# Autodesk Inventor assembly: GabelTop_Link_COG
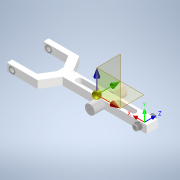
[picture p0: Inventor's stored thumbnail of the model, 180x180]
Saved by Autodesk Inventor 2022 (Build 260153000, 153)
## iProperties
Created: 2022-10-18
Part Number: GabelTop_Link_COG
Document SubType Name: Assembly
Designer: alexw
Mass: 378.635 g
Surface Area: 728.449 cm^2
Volume: 214.913 cm^3
Density: 1.7618 g/cm^3
Author: alexw
## Documents named in this file (5)
- C:\Users\alexw\Documents\Inventor\Projects\03_CurrentProjects\MasterThesis\PSM_V1_Rillenkugellager\COG\GabelTop_Link_COG.iam
- C:\Users\alexw\Documents\Inventor\Projects\03_CurrentProjects\MasterThesis\PSM_V1_Rillenkugellager\Adaptationhorizontalachse_Assembly_Rillenkugellager.iam
- C:\Users\alexw\Documents\Inventor\Projects\03_CurrentProjects\MasterThesis\PSM_V1_Rillenkugellager\SpringCompensation_Outside_SupportPart.ipt
- C:\Users\alexw\Documents\Inventor\Projects\03_CurrentProjects\MasterThesis\PSM_V1_Rillenkugellager\SpringCompensation_Outside_SupportPart_Zwischenstueck.ipt
- C:\Users\alexw\Documents\Inventor\Projects\03_CurrentProjects\MasterThesis\PSM_V1_Rillenkugellager\ContentCenter\de-DE\ISO 4762(2)\ISO 4762 - M10 x 20ISO.ipt
## Components (7 placed, 4 different names)
1. Adaptationhorizontalachse_Assembly_Rillenkugellager:1 [sub-assembly] — Passend:9, Passend:10, Winkel:1, Passend:11, Passend:12, Passend:13, Passend:14, Passend:15, Passend:16, Passend:18
2. SpringCompensation_Outside_SupportPart:1 — Passend:20, Passend:21
3. SpringCompensation_Outside_SupportPart_Zwischenstueck:1 — Passend:12, Passend:13, Passend:17, Passend:20, Passend:21
4. SpringCompensation_Outside_SupportPart_Zwischenstueck:2 — Passend:14, Passend:15, Passend:19, Passend:22, Passend:23
5. ISO 4762 M10 x 20:1 — Passend:16, Passend:17
6. ISO 4762 M10 x 20:2 — Passend:18, Passend:19
7. SpringCompensation_Outside_SupportPart:2 — Passend:22, Passend:23
## Relationships (16: Mate 15, Angle 1)
- Passend:9 [Mate]: Adaptationhorizontalachse_Assembly_Rillenkugellager:1
- Passend:10 [Mate]: Adaptationhorizontalachse_Assembly_Rillenkugellager:1
- Winkel:1 [Angle] (0 deg): Adaptationhorizontalachse_Assembly_Rillenkugellager:1
- Passend:11 [Mate]: Adaptationhorizontalachse_Assembly_Rillenkugellager:1
- Passend:12 [Mate]: Adaptationhorizontalachse_Assembly_Rillenkugellager:1 ↔ SpringCompensation_Outside_SupportPart_Zwischenstueck:1
- Passend:13 [Mate]: Adaptationhorizontalachse_Assembly_Rillenkugellager:1 ↔ SpringCompensation_Outside_SupportPart_Zwischenstueck:1
- Passend:14 [Mate]: Adaptationhorizontalachse_Assembly_Rillenkugellager:1 ↔ SpringCompensation_Outside_SupportPart_Zwischenstueck:2
- Passend:15 [Mate]: Adaptationhorizontalachse_Assembly_Rillenkugellager:1 ↔ SpringCompensation_Outside_SupportPart_Zwischenstueck:2
- Passend:16 [Mate]: Adaptationhorizontalachse_Assembly_Rillenkugellager:1 ↔ ISO 4762 M10 x 20:1
- Passend:17 [Mate]: SpringCompensation_Outside_SupportPart_Zwischenstueck:1 ↔ ISO 4762 M10 x 20:1
- Passend:18 [Mate]: Adaptationhorizontalachse_Assembly_Rillenkugellager:1 ↔ ISO 4762 M10 x 20:2
- Passend:19 [Mate]: SpringCompensation_Outside_SupportPart_Zwischenstueck:2 ↔ ISO 4762 M10 x 20:2
- Passend:20 [Mate]: SpringCompensation_Outside_SupportPart:1 ↔ SpringCompensation_Outside_SupportPart_Zwischenstueck:1
- Passend:21 [Mate]: SpringCompensation_Outside_SupportPart:1 ↔ SpringCompensation_Outside_SupportPart_Zwischenstueck:1
- Passend:22 [Mate]: SpringCompensation_Outside_SupportPart_Zwischenstueck:2 ↔ SpringCompensation_Outside_SupportPart:2
- Passend:23 [Mate]: SpringCompensation_Outside_SupportPart_Zwischenstueck:2 ↔ SpringCompensation_Outside_SupportPart:2
